# Autodesk Inventor assembly: SmolAssembly
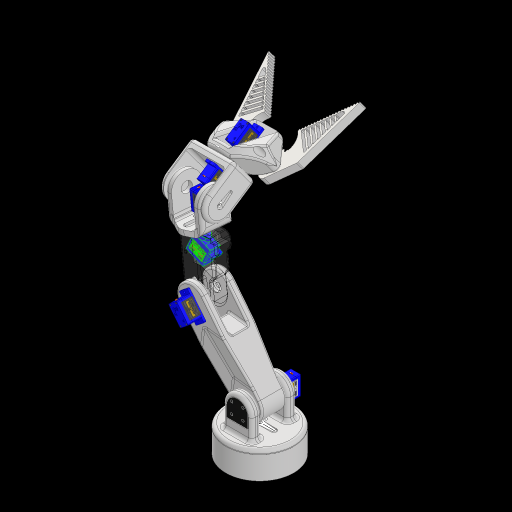
[picture p0: Inventor's stored thumbnail of the model, 512x512]
Saved by Autodesk Inventor 2023 (Build 270158000, 158)
## iProperties
Created: 2023-05-15
Part Number: SmolAssembly
Document SubType Name: Assembly
Designer: tandu
Author: tandu
## Documents named in this file (10)
- C:\Users\tandu\Documents\GrabCAD\Robotic Arm Project\Smol Version\V1\SmolAssembly.iam
- C:\Users\tandu\Documents\GrabCAD\Robotic Arm Project\Smol Version\V1\Base.ipt
- C:\Users\tandu\Documents\GrabCAD\Robotic Arm Project\Smol Version\V1\SG90 Assembly.iam
- C:\Users\tandu\Documents\GrabCAD\Robotic Arm Project\Smol Version\V1\FirstJoint.ipt
- C:\Users\tandu\Documents\GrabCAD\Robotic Arm Project\Smol Version\V1\FirstLink.ipt
- C:\Users\tandu\Documents\GrabCAD\Robotic Arm Project\Smol Version\V1\SecondJoint.ipt
- C:\Users\tandu\Documents\GrabCAD\Robotic Arm Project\Smol Version\V1\ThirdJoint.ipt
- C:\Users\tandu\Documents\GrabCAD\Robotic Arm Project\Smol Version\V1\FourthJoint.ipt
- C:\Users\tandu\Documents\GrabCAD\Robotic Arm Project\Smol Version\V1\Claw\SmolClawAssembly.iam
- C:\Users\tandu\Documents\GrabCAD\Robotic Arm Project\Smol Version\V1\FirstJointAxle.ipt
## Components (15 placed, 9 different names)
1. Base:1 — Insert:1, Insert:2, Insert:3
2. SG90 Assembly:1 [sub-assembly] — Insert:1, Insert:2, Angle:1
3. FirstJoint:1 — Insert:3, Angle:1, Insert:17, Insert:18, Insert:19, Insert:20
4. SG90 Assembly:2 [sub-assembly] — Mate:1, Mate:2, Insert:19, Insert:20
5. FirstLink:1 — Mate:1, Mate:2, Mate:4, Insert:15, Insert:16
6. SG90 Assembly:3 [sub-assembly] — Mate:3, Insert:15, Insert:16
7. SecondJoint:1 — Mate:3, Mate:4, Insert:21, Insert:22, Mate:9, Mate:10
8. SG90 Assembly:4 [sub-assembly] — Mate:5, Mate:6, Insert:21, Insert:22
9. ThirdJoint:1 — Mate:5, Mate:6, Insert:10, Insert:11
10. SG90 Assembly:5 [sub-assembly] — Insert:10, Insert:11, Mate:7, Mate:8
11. FourthJoint:1 — Mate:7, Mate:8, Insert:12, Insert:13, Angle:2
12. SG90 Assembly:6 [sub-assembly] — Insert:12, Insert:13, Insert:14
13. SmolClawAssembly:1 [sub-assembly] — Insert:14, Angle:2
14. FirstJointAxle:1 — Insert:17, Insert:18
15. SG90 Assembly:7 [sub-assembly] — Mate:9, Mate:10
## Relationships (28: Insert 16, Mate 10, Angle 2)
- Insert:1: Base:1 ↔ SG90 Assembly:1
- Insert:2: Base:1 ↔ SG90 Assembly:1
- Insert:3: Base:1 ↔ FirstJoint:1
- Angle:1 (180 deg): SG90 Assembly:1 ↔ FirstJoint:1
- Mate:1: SG90 Assembly:2 ↔ FirstLink:1
- Mate:2: SG90 Assembly:2 ↔ FirstLink:1
- Mate:3: SG90 Assembly:3 ↔ SecondJoint:1
- Mate:4: FirstLink:1 ↔ SecondJoint:1
- Mate:5: SG90 Assembly:4 ↔ ThirdJoint:1
- Mate:6: SG90 Assembly:4 ↔ ThirdJoint:1
- Insert:10: ThirdJoint:1 ↔ SG90 Assembly:5
- Insert:11: ThirdJoint:1 ↔ SG90 Assembly:5
- Mate:7: SG90 Assembly:5 ↔ FourthJoint:1
- Mate:8: SG90 Assembly:5 ↔ FourthJoint:1
- Insert:12: FourthJoint:1 ↔ SG90 Assembly:6
- Insert:13: FourthJoint:1 ↔ SG90 Assembly:6
- Insert:14: SG90 Assembly:6 ↔ SmolClawAssembly:1
- Angle:2 (180 deg): FourthJoint:1 ↔ SmolClawAssembly:1
- Insert:15: FirstLink:1 ↔ SG90 Assembly:3
- Insert:16: FirstLink:1 ↔ SG90 Assembly:3
- Insert:17: FirstJoint:1 ↔ FirstJointAxle:1
- Insert:18: FirstJoint:1 ↔ FirstJointAxle:1
- Insert:19: FirstJoint:1 ↔ SG90 Assembly:2
- Insert:20: FirstJoint:1 ↔ SG90 Assembly:2
- Insert:21: SecondJoint:1 ↔ SG90 Assembly:4
- Insert:22: SecondJoint:1 ↔ SG90 Assembly:4
- Mate:9: SecondJoint:1 ↔ SG90 Assembly:7
- Mate:10: SecondJoint:1 ↔ SG90 Assembly:7
